# Autodesk Inventor assembly: socket
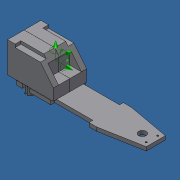
[picture p0: Inventor's stored thumbnail of the model, 180x180]
Saved by Autodesk Inventor 2022.4 (Build 264492010, 492A)
## iProperties
Created: 2005-04-19
Part Number: socket
Document SubType Name: Assembly
Designer: skovacevic
Manufacturer: Standard
Standards Organization: Custom
Mass: 2.81525 g
Surface Area: 35.2605 cm^2
Volume: 2.81525 cm^3
Density: 1 g/cm^3
CN_MASS: 0
Author: skovacevic
## Documents named in this file (7)
- U:\Inventor 2022 Training\_Designer Training\Inventor 2022 - Advanced Assembly\Practice Files\Mirror Assembly Components\socket.iam
- U:\Inventor 2022 Training\_Designer Training\Inventor 2022 - Advanced Assembly\Practice Files\Mirror Assembly Components\encbase.ipt
- U:\Inventor 2022 Training\_Designer Training\Inventor 2022 - Advanced Assembly\Practice Files\Mirror Assembly Components\pcb.ipt
- U:\Inventor 2022 Training\_Designer Training\Inventor 2022 - Advanced Assembly\Practice Files\Mirror Assembly Components\connect.ipt
- U:\Inventor 2022 Training\_Designer Training\Inventor 2022 - Advanced Assembly\Practice Files\Mirror Assembly Components\wire.ipt
- U:\Inventor 2022 Training\_Designer Training\Inventor 2022 - Advanced Assembly\Practice Files\Mirror Assembly Components\enctop.ipt
- U:\Inventor 2022 Training\_Designer Training\Inventor 2022 - Advanced Assembly\Practice Files\Mirror Assembly Components\connect_MIR.ipt
## Components (6 placed, 6 different names)
1. encbase:1 — Insert:1, Angle:1, Insert:3, Mate:1, Flush:1, Flush:2, Mate:2
2. pcb:1 — Insert:1, Angle:1, Angle:2, Insert:2
3. connect:1 — Angle:2, Insert:2
4. wire:1 — Insert:3, Mate:1
5. enctop:1 — Flush:1, Flush:2, Mate:2
6. connect_MIR:1
## Relationships (9: Insert 3, Angle 2, Mate 2, Flush 2)
- Insert:1 (-6.985 mm): encbase:1 ↔ pcb:1
- Angle:1 (180 deg): encbase:1 ↔ pcb:1
- Angle:2 (0 deg): pcb:1 ↔ connect:1
- Insert:2: pcb:1 ↔ connect:1
- Insert:3: encbase:1 ↔ wire:1
- Mate:1: encbase:1 ↔ wire:1
- Flush:1: encbase:1 ↔ enctop:1
- Flush:2: encbase:1 ↔ enctop:1
- Mate:2: encbase:1 ↔ enctop:1
